# Autodesk Inventor assembly: LimitSwitchAssembly
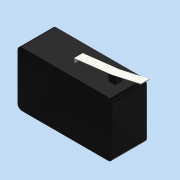
[picture p0: Inventor's stored thumbnail of the model, 180x180]
Saved by Autodesk Inventor 2017 (Build 210142000, 142)
## iProperties
Created: 2016-12-03
Part Number: LimitSwitchAssembly
Document SubType Name: Assembly
Designer: techn
Author: techn
## Documents named in this file (3)
- D:\OneDrive\Documents\Other Projects\Submarine\CAD\common\Switches\LimitSwitch\LimitSwitchAssembly.iam
- D:\OneDrive\Documents\Other Projects\Submarine\CAD\common\Switches\LimitSwitch\LIMIT SWITCH.ipt
- D:\OneDrive\Documents\Other Projects\Submarine\CAD\common\Switches\LimitSwitch\limitSwitchTrigger.ipt
## Components (2 placed, 2 different names)
1. LIMIT SWITCH:1 — Mate:1, Flush:1
2. limitSwitchTrigger:1 — Mate:1, Flush:1
## Relationships (2: Mate 1, Flush 1)
- Mate:1: LIMIT SWITCH:1 ↔ limitSwitchTrigger:1
- Flush:1 (3.81 mm): LIMIT SWITCH:1 ↔ limitSwitchTrigger:1
